# Autodesk Inventor assembly: asmTemp
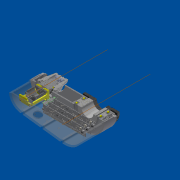
[picture p0: Inventor's stored thumbnail of the model, 180x180]
Saved by Autodesk Inventor 2018 (Build 220112000, 112)
## iProperties
Created: 2019-11-13
Part Number: asmTemp
Document SubType Name: Assembly
Designer: Bunny320
Author: Bunny320
## Documents named in this file (17)
- C:\Users\Bunny320\Desktop\sechs\4-CAD\10-J1.iam
- C:\Users\Bunny320\Desktop\sechs\4-CAD\generated\J1_belt.iam
- C:\Users\Bunny320\Desktop\sechs\4-CAD\standardParts\61814-2RS1\61814-2RS1.iam
- C:\Users\Bunny320\Desktop\sechs\4-CAD\105-flange adapter.ipt
- C:\Users\Bunny320\Documents\Inventor\Content Center Files\R2018\en-US\ISO 10642(2)\ISO 10642  - M3  x  20.ipt
- C:\Users\Bunny320\Documents\Inventor\Content Center Files\R2018\en-US\ISO 4762(1)\DIN EN ISO 4762 - M2 x 6.ipt
- C:\Users\Bunny320\Documents\Inventor\Content Center Files\R2018\en-US\DIN EN ISO 4032\DIN EN ISO 4032 - M2.ipt
- C:\Users\Bunny320\Documents\Inventor\Content Center Files\R2018\en-US\ISO 4762(1)\DIN EN ISO 4762 - M3 x 10.ipt
- C:\Users\Bunny320\Desktop\sechs\4-CAD\standardParts\Pololu mounting hub\pololu-universal-aluminum-mounting-hub-for-6mm-shaft-m3-holes.ipt
- C:\Users\Bunny320\Desktop\sechs\4-CAD\standardParts\61807-2RS1\61807-2RS1.iam
- C:\Users\Bunny320\Desktop\sechs\4-CAD\generated\J1_belt\Design Accelerator\Synchronous Pulley11.ipt
- C:\Users\Bunny320\Desktop\sechs\4-CAD\standardParts\Odrive\PCBasembly_simp.ipt
- C:\Users\Bunny320\Desktop\sechs\4-CAD\motor unit 2820 (J1).iam
- C:\Users\Bunny320\Desktop\sechs\4-CAD\106-pulley adapter.ipt
- C:\Users\Bunny320\Desktop\sechs\4-CAD\112-base middle.ipt
- C:\Users\Bunny320\Desktop\sechs\4-CAD\113-base bottom.ipt
- C:\Users\Bunny320\Desktop\sechs\4-CAD\114-base top.ipt
## Components (40 placed, 16 different names)
1. 112-base middle:1 — Mate:5, Mate:102, Mate:107, Mate:108, Mate:109, Mate:111, Mate:112, Mate:113
2. J1_belt:1 [sub-assembly] — Mate:1, Mate:2, Mate:3, Mate:6, Mate:7, Mate:8, Mate:30, Mate:32, Mate:33, Mate:34, Mate:35, Mate:101, Mate:105, Mate:106
3. 61814-2RS1:1 [sub-assembly] — Mate:2, Mate:8, Mate:110
4. 61814-2RS1:2 [sub-assembly] — Mate:3, Mate:5, Mate:7
5. 105-flange adapter:1 — Mate:30, Mate:105, Mate:106
6. DIN EN ISO 10642 M3  x  20:1 — Mate:32
7. DIN EN ISO 10642 M3  x  20:2 — Mate:33
8. DIN EN ISO 10642 M3  x  20:3 — Mate:34
9. DIN EN ISO 10642 M3  x  20:4 — Mate:35
10. DIN EN ISO 4762 M2 x 6:1 — Mate:50
11. DIN EN ISO 4762 M2 x 6:2 — Mate:46
12. DIN EN ISO 4762 M2 x 6:3 — Mate:44
13. DIN EN ISO 4762 M2 x 6:4 — Mate:48
14. DIN EN ISO 4032 M2:1 — Mate:44
15. DIN EN ISO 4032 M2:2 — Mate:46
16. DIN EN ISO 4032 M2:3 — Mate:48
17. DIN EN ISO 4032 M2:4 — Mate:50
18. DIN EN ISO 4762 M3 x 10:1
19. DIN EN ISO 4762 M3 x 10:2
20. DIN EN ISO 4762 M3 x 10:3
21. DIN EN ISO 4762 M3 x 10:4
22. DIN EN ISO 4762 M3 x 10:5
23. DIN EN ISO 4762 M3 x 10:6
24. DIN EN ISO 4762 M3 x 10:7
25. DIN EN ISO 4762 M3 x 10:8
26. DIN EN ISO 4762 M3 x 10:9
27. DIN EN ISO 4762 M3 x 10:10
28. DIN EN ISO 4762 M3 x 10:11
29. DIN EN ISO 4762 M3 x 10:12
30. DIN EN ISO 4762 M3 x 10:13
31. motor unit 2820 (J1):1 [sub-assembly] — Flush:4, Mate:92, Mate:100, Mate:101, Mate:102
32. pololu-universal-aluminum-mounting-hub-for-6mm-shaft-m3-holes:1 — Flush:4, Mate:92, Mate:97
33. 61807-2RS1:1 [sub-assembly] — Mate:98, Mate:99, Mate:100, Mate:103, Mate:104
34. Synchronous Pulley1:1 — Mate:97, Mate:98, Mate:99
35. PCBasembly_simp:1 — Mate:112, Mate:113
36. 106-pulley adapter:1 — Mate:103, Mate:104
37. 113-base bottom:1 — Mate:107, Mate:108, Mate:109
38. 114-base top:1 — Mate:110, Mate:111
39. PCBasembly_simp:2
40. PCBasembly_simp:3
## Relationships (38: Mate 34, Flush 4)
- [Flush]: 112-base middle:1
- [Flush]: 112-base middle:1
- [Flush]: 112-base middle:1
- Mate:1: J1_belt:1
- Mate:2: J1_belt:1 ↔ 61814-2RS1:1
- Mate:3: J1_belt:1 ↔ 61814-2RS1:2
- Mate:5: 112-base middle:1 ↔ 61814-2RS1:2
- Mate:6: J1_belt:1
- Mate:7: J1_belt:1 ↔ 61814-2RS1:2
- Mate:8: J1_belt:1 ↔ 61814-2RS1:1
- Mate:30: J1_belt:1 ↔ 105-flange adapter:1
- Mate:32: J1_belt:1 ↔ DIN EN ISO 10642 M3  x  20:1
- Mate:33: J1_belt:1 ↔ DIN EN ISO 10642 M3  x  20:2
- Mate:34: J1_belt:1 ↔ DIN EN ISO 10642 M3  x  20:3
- Mate:35: J1_belt:1 ↔ DIN EN ISO 10642 M3  x  20:4
- Mate:44: DIN EN ISO 4762 M2 x 6:3 ↔ DIN EN ISO 4032 M2:1
- Mate:46: DIN EN ISO 4762 M2 x 6:2 ↔ DIN EN ISO 4032 M2:2
- Mate:48: DIN EN ISO 4762 M2 x 6:4 ↔ DIN EN ISO 4032 M2:3
- Mate:50: DIN EN ISO 4762 M2 x 6:1 ↔ DIN EN ISO 4032 M2:4
- Flush:4: motor unit 2820 (J1):1 ↔ pololu-universal-aluminum-mounting-hub-for-6mm-shaft-m3-holes:1
- Mate:92: motor unit 2820 (J1):1 ↔ pololu-universal-aluminum-mounting-hub-for-6mm-shaft-m3-holes:1
- Mate:97: pololu-universal-aluminum-mounting-hub-for-6mm-shaft-m3-holes:1 ↔ Synchronous Pulley1:1
- Mate:98: 61807-2RS1:1 ↔ Synchronous Pulley1:1
- Mate:99: 61807-2RS1:1 ↔ Synchronous Pulley1:1
- Mate:100: motor unit 2820 (J1):1 ↔ 61807-2RS1:1
- Mate:101: J1_belt:1 ↔ motor unit 2820 (J1):1
- Mate:102: 112-base middle:1 ↔ motor unit 2820 (J1):1
- Mate:103: 61807-2RS1:1 ↔ 106-pulley adapter:1
- Mate:104: 61807-2RS1:1 ↔ 106-pulley adapter:1
- Mate:105: J1_belt:1 ↔ 105-flange adapter:1
- Mate:106: J1_belt:1 ↔ 105-flange adapter:1
- Mate:107: 112-base middle:1 ↔ 113-base bottom:1
- Mate:108: 112-base middle:1 ↔ 113-base bottom:1
- Mate:109: 112-base middle:1 ↔ 113-base bottom:1
- Mate:110: 61814-2RS1:1 ↔ 114-base top:1
- Mate:111: 112-base middle:1 ↔ 114-base top:1
- Mate:112: 112-base middle:1 ↔ PCBasembly_simp:1
- Mate:113: 112-base middle:1 ↔ PCBasembly_simp:1
